# Autodesk Inventor assembly: Zusammenbau_Gruppe7
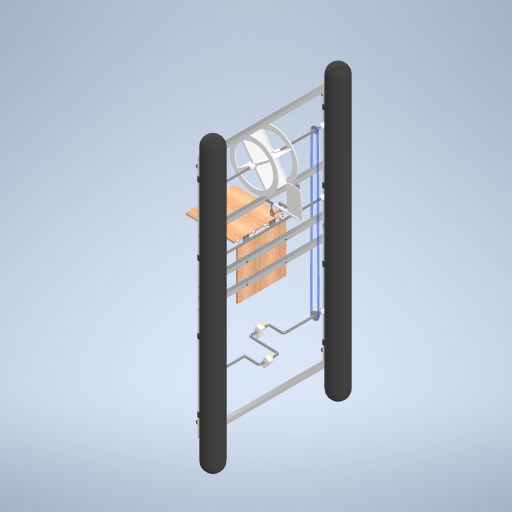
[picture p0: Inventor's stored thumbnail of the model, 512x512]
Saved by Autodesk Inventor 2024.4 (Build 284460000, 460)
## iProperties
Created: 2026-01-14
Part Number: Zusammenbau_Gruppe7
Description: Zusammenbau
Document SubType Name: Assembly
Designer: Philf
Mass: 49081.2 g
Surface Area: 141619 cm^2
Volume: 28441.6 cm^3
Density: 1.72568 g/cm^3
Masse[kg]: 49,1 kg
## Documents named in this file (35)
- C:\Users\Philf\Documents\Vault\Daten\I60-Konstruktion\I60-Gruppe-7\Konzept\Teil2\Zusammenbau_Gruppe7.iam
- C:\Users\Philf\Documents\Vault\Daten\I60-Konstruktion\I60-Gruppe-7\Gestell\Gestell_zsm.iam
- C:\Users\Philf\Documents\Vault\Daten\I60-Konstruktion\I60-Gruppe-7\Schwimmkoerper\Schwimmkoerper.iam
- C:\Users\Philf\Documents\Vault\Daten\I60-Konstruktion\I60-Gruppe-7\schaufelrad\Schaufelrad.iam
- C:\Users\Philf\Documents\Vault\Daten\I60-Konstruktion\I60-Gruppe-7\Tritt\Stange.iam
- C:\Users\Philf\Documents\Vault\Daten\I60-Konstruktion\I60-Gruppe-7\Tritt\Pedale.iam
- C:\Users\Philf\Documents\Vault\Daten\I60-Konstruktion\I60-Gruppe-7\Sitz\sitz_zusammenbau.iam
- C:\Users\Philf\Documents\Vault\Normteile\de-DE\DIN EN ISO 4032\DIN EN ISO 4032 - M10.ipt
- C:\Users\Philf\Documents\Vault\Normteile\de-DE\ISO 10642(2)\ISO 10642  - M10  x  70.ipt
- C:\Users\Philf\Documents\Vault\Daten\I60-Konstruktion\I60-Gruppe-7\Tritt\stopper2.ipt
- C:\Users\Philf\Documents\Vault\Normteile\de-DE\ISO 4762(1)\DIN EN ISO 4762 - M5 x 20.ipt
- C:\Users\Philf\Documents\Vault\Daten\I60-Konstruktion\I60-Gruppe-7\Tritt\6799K141_Machinable-Bore Corrosion-Resistant Sprocket.ipt
- C:\Users\Philf\Documents\Vault\Normteile\de-DE\ISO 4762(1)\DIN EN ISO 4762 - M10 x 60.ipt
- C:\Users\Philf\Documents\Vault\Normteile\de-DE\ISO 4762(1)\DIN EN ISO 4762 - M5 x 16.ipt
- C:\Users\Philf\Documents\Vault\Daten\I60-Konstruktion\I60-Gruppe-7\Tritt\6799K144_Machinable-Bore Corrosion-Resistant Sprocket\6799K144_Machinable-Bore Corrosion-Resistant Sprocket\6799K144_Machinable-Bore Corr.ipt
- C:\Users\Philf\Documents\Vault\Daten\I60-Konstruktion\I60-Gruppe-7\Zusammenbau\Konstruktions-Assistent\HTW-000642.iam
- C:\Users\Philf\Documents\Vault\Daten\I60-Konstruktion\I60-Gruppe-7\schaufelrad\Stangeschaufelrad.ipt
- C:\Users\Philf\Documents\Vault\Daten\I60-Konstruktion\I60-Gruppe-7\Steuern\HTW-000654.ipt
- C:\Users\Philf\Documents\Vault\Daten\I60-Konstruktion\I60-Gruppe-7\Steuern\Verbindung.ipt
- C:\Users\Philf\Documents\Vault\Daten\I60-Konstruktion\I60-Gruppe-7\Steuern\ustück.ipt
- C:\Users\Philf\Documents\Vault\Daten\I60-Konstruktion\I60-Gruppe-7\Steuern\clevisPin30.ipt
- C:\Users\Philf\Documents\Vault\Daten\I60-Konstruktion\I60-Gruppe-7\Steuern\cotterpin.ipt
- C:\Users\Philf\Documents\Vault\Daten\I60-Konstruktion\I60-Gruppe-7\Steuern\HTW-000679.ipt
- C:\Users\Philf\Documents\Vault\Daten\I60-Konstruktion\I60-Gruppe-7\Steuern\HTW-000681.ipt
- C:\Users\Philf\Documents\Vault\Daten\I60-Konstruktion\I60-Gruppe-7\Steuern\Rod End Nuts.ipt
- C:\Users\Philf\Documents\Vault\Daten\I60-Konstruktion\I60-Gruppe-7\Steuern\steuerstange.ipt
- C:\Users\Philf\Documents\Vault\Daten\I60-Konstruktion\I60-Gruppe-7\Steuern\HTW-000692.ipt
- C:\Users\Philf\Documents\Vault\Daten\I60-Konstruktion\I60-Gruppe-7\Gestell\richtungstange.ipt
- C:\Users\Philf\Documents\Vault\Daten\I60-Konstruktion\I60-Gruppe-7\Steuern\HTW-000702.ipt
- C:\Users\Philf\Documents\Vault\Normteile\de-DE\DIN EN ISO 7093-1\DIN EN ISO 7093-1 - 8.ipt
- C:\Users\Philf\Documents\Vault\Daten\I60-Konstruktion\I60-Gruppe-7\Gestell\LagerBund.ipt
- C:\Users\Philf\Documents\Vault\Normteile\de-DE\ISO 4762(1)\DIN EN ISO 4762 - M8 x 16.ipt
- C:\Users\Philf\Documents\Vault\Normteile\de-DE\ISO 4762(1)\DIN EN ISO 4762 - M8 x 25.ipt
- C:\Users\Philf\Documents\Vault\Normteile\de-DE\ISO 4762(1)\DIN EN ISO 4762 - M5 x 25.ipt
- C:\Users\Philf\Documents\Vault\Normteile\de-DE\ISO 4762(1)\DIN EN ISO 4762 - M5 x 8.ipt
## Components (98 placed, 34 different names)
1. Gestell_zsm:1 [sub-assembly] — Passend:1, Passend:2, Passend:3, Passend:4, Passend:5, Passend:6, Passend:7, Passend:8, Passend:9, Drehbar:1, Drehbar:4, Passend:12, Passend:13, Passend:14, Einfügen:1, Einfügen:2, Einfügen:3, Einfügen:4, Passend:24, Passend:26, Einfügen:9, Einfügen:10, Einfügen:11, Einfügen:12, Einfügen:13, Einfügen:14, Einfügen:15, Einfügen:16, Einfügen:17, Einfügen:18, Einfügen:19, Einfügen:20, Einfügen:29, Einfügen:30, Einfügen:31, Einfügen:32, Einfügen:33, Einfügen:34, Einfügen:35, Einfügen:36, Einfügen:37, Einfügen:38, Einfügen:39, Einfügen:40, Fluchtend:2, Passend:32, Fluchtend:3, Passend:70, Passend:74, Fluchtend:5, Passend:75, Passend:102, Passend:104, Einfügen:55, Einfügen:56
2. Schwimmkoerper:1 [sub-assembly] — Passend:5, Passend:7, Passend:8, Winkel:1
3. Schwimmkoerper:2 [sub-assembly] — Passend:4, Passend:6, Passend:9, Winkel:2, Fluchtend:2
4. Schaufelrad:1 [sub-assembly] — Drehbar:4, Passend:23, Passend:25, Winkel:3, Winkel:4, Passend:27, Passend:29
5. Stange:1 [sub-assembly] — Drehbar:1, Drehbar:2, Drehbar:3, Passend:10, Passend:11, Einfügen:21, Einfügen:22, Einfügen:23, Einfügen:24, Passend:30, Passend:31, Winkel:5
6. Pedale:1 [sub-assembly] — Drehbar:2, Passend:10
7. Pedale:2 [sub-assembly] — Drehbar:3, Passend:11
8. sitz_zusammenbau:1 [sub-assembly] — Passend:12, Passend:13, Passend:14, Passend:15, Passend:16, Passend:17, Passend:18
9. DIN EN ISO 4032 M10:1 — Einfügen:1
10. DIN EN ISO 4032 M10:2 — Einfügen:2
11. DIN EN ISO 4032 M10:3 — Einfügen:3
12. DIN EN ISO 4032 M10:4 — Einfügen:4
13. DIN EN ISO 10642 M10  x  70:1 — Passend:15
14. DIN EN ISO 10642 M10  x  70:2 — Passend:16
15. DIN EN ISO 10642 M10  x  70:3 — Passend:17
16. DIN EN ISO 10642 M10  x  70:4 — Passend:18
17. stopper2:1 — Passend:23, Passend:24, Winkel:4, Einfügen:5, Einfügen:6
18. stopper2:2 — Passend:25, Passend:26, Winkel:3, Einfügen:7, Einfügen:8
19. DIN EN ISO 4762 M5 x 20:1 — Einfügen:5
20. DIN EN ISO 4762 M5 x 20:2 — Einfügen:6
21. DIN EN ISO 4762 M5 x 20:3 — Einfügen:7
22. DIN EN ISO 4762 M5 x 20:4 — Einfügen:8
23. 6799K141_Machinable-Bore Corrosion-Resistant Sprocket:1 — Passend:27, Passend:29, Einfügen:28, Fluchtend:1, Drehung:1
24. DIN EN ISO 4762 M10 x 60:1 — Einfügen:9
25. DIN EN ISO 4762 M10 x 60:2 — Einfügen:10
26. DIN EN ISO 4762 M10 x 60:3 — Einfügen:11
27. DIN EN ISO 4762 M10 x 60:4 — Einfügen:12
28. DIN EN ISO 4762 M10 x 60:5 — Einfügen:13
29. DIN EN ISO 4762 M10 x 60:6 — Einfügen:14
30. DIN EN ISO 4762 M10 x 60:7 — Einfügen:15
31. DIN EN ISO 4762 M10 x 60:8 — Einfügen:16
32. DIN EN ISO 4762 M10 x 60:9 — Einfügen:17
33. DIN EN ISO 4762 M10 x 60:10 — Einfügen:18
34. DIN EN ISO 4762 M10 x 60:11 — Einfügen:19
35. DIN EN ISO 4762 M10 x 60:12 — Einfügen:20
36. DIN EN ISO 4762 M5 x 20:5 — Einfügen:21
37. DIN EN ISO 4762 M5 x 20:6 — Einfügen:22
38. DIN EN ISO 4762 M5 x 20:7 — Einfügen:23
39. DIN EN ISO 4762 M5 x 20:8 — Einfügen:24
40. DIN EN ISO 4762 M5 x 16:4 — Einfügen:28
41. DIN EN ISO 4032 M10:5 — Einfügen:29
42. DIN EN ISO 4032 M10:6 — Einfügen:30
43. DIN EN ISO 4032 M10:7 — Einfügen:31
44. DIN EN ISO 4032 M10:8 — Einfügen:32
45. DIN EN ISO 4032 M10:9 — Einfügen:33
46. DIN EN ISO 4032 M10:10 — Einfügen:34
47. DIN EN ISO 4032 M10:11 — Einfügen:35
48. DIN EN ISO 4032 M10:12 — Einfügen:36
49. DIN EN ISO 4032 M10:13 — Einfügen:37
50. DIN EN ISO 4032 M10:14 — Einfügen:38
51. DIN EN ISO 4032 M10:15 — Einfügen:39
52. DIN EN ISO 4032 M10:16 — Einfügen:40
53. 6799K144_Machinable-Bore Corr:1 — Passend:30, Passend:31, Fluchtend:1, Winkel:5, Drehung:1, Einfügen:41
54. Kettenantrieb:1 [sub-assembly]
55. DIN EN ISO 4762 M5 x 16:5 — Einfügen:41
56. Stangeschaufelrad:1 — Passend:32, Fluchtend:3, Passend:33, Passend:101, Passend:103
57. HTW-000654:1 — Passend:90, Passend:91, Fluchtend:11, Passend:105, Passend:106
58. Verbindung:1 — Passend:33, Passend:70, Einfügen:48, Einfügen:49, Einfügen:50, Fluchtend:11, Passend:105, Passend:106
59. ustück:1 — Passend:37, Passend:38, Passend:87, Passend:88, Passend:91
60. clevisPin30:1 — Passend:37, Passend:38, Passend:39, Passend:41, Passend:90
61. cotterpin:1 — Passend:39, Passend:41
62. ustück:2 — Passend:48, Passend:49, Passend:82, Passend:85, Passend:86
63. clevisPin30:2 — Passend:48, Passend:49, Passend:81
64. cotterpin:2
65. HTW-000681:1 — Passend:50, Passend:51, Passend:56, Passend:57, Passend:76, Passend:77, Passend:97, Fluchtend:9, Einfügen:43
66. Rod End Nuts:1 — Passend:50, Passend:51, Passend:81, Passend:82
67. ustück:3 — Passend:56, Passend:57, Passend:95
68. clevisPin30:3 — Passend:94
69. cotterpin:3
70. Rod End Nuts:2 — Passend:58, Passend:59, Passend:94, Passend:95
71. HTW-000679:2 — Passend:58, Passend:59, Passend:66, Passend:67
72. ustück:4 — Passend:68, Passend:69, Passend:93
73. clevisPin30:4 — Passend:92
74. cotterpin:4
75. Rod End Nuts:4 — Passend:66, Passend:67, Passend:92, Passend:93
76. steuerstange:1 — Passend:68, Passend:69, Passend:71, Passend:72, Passend:73, Passend:83, Passend:84, Passend:96, Fluchtend:10, Einfügen:42
77. HTW-000692:1 — Passend:71, Passend:72, Passend:73, Winkel:6, Einfügen:46, Einfügen:47
78. richtungstange:1 — Passend:74, Fluchtend:5, Passend:75, Passend:76, Passend:77, Passend:83, Passend:84, Passend:98, Passend:99
79. HTW-000702:1 — Passend:85, Passend:86, Passend:87, Passend:88
80. LagerBund:1 — Passend:97, Passend:98, Fluchtend:9
81. LagerBund:2 — Passend:96, Passend:99, Fluchtend:10
82. DIN EN ISO 7093-1 8:1 — Einfügen:42, Einfügen:45
83. DIN EN ISO 7093-1 8:2 — Einfügen:43, Einfügen:44
84. DIN EN ISO 4762 M8 x 16:1 — Einfügen:44
85. DIN EN ISO 4762 M8 x 16:2 — Einfügen:45
86. DIN EN ISO 4762 M8 x 25:1 — Einfügen:46
87. DIN EN ISO 4762 M8 x 25:2 — Einfügen:47
88. DIN EN ISO 4762 M5 x 25:1 — Einfügen:48
89. DIN EN ISO 4762 M5 x 8:1 — Einfügen:49
90. DIN EN ISO 4762 M5 x 8:2 — Einfügen:50
91. stopper2:3 — Passend:103, Passend:104, Einfügen:51, Einfügen:52
92. stopper2:4 — Passend:101, Passend:102, Einfügen:53, Einfügen:54
93. DIN EN ISO 4762 M5 x 20:9 — Einfügen:51
94. DIN EN ISO 4762 M5 x 20:10 — Einfügen:52
95. DIN EN ISO 4762 M5 x 20:11 — Einfügen:53
96. DIN EN ISO 4762 M5 x 20:12 — Einfügen:54
97. DIN EN ISO 4762 M10 x 60:13 — Einfügen:55
98. DIN EN ISO 4762 M10 x 60:14 — Einfügen:56
## Relationships (157: Mate 86, Insert 53, Flush 7, Angle 6, RevoluteJoint 4, RelateRotation 1)
- Passend:1 [Mate]: Gestell_zsm:1
- Passend:2 [Mate]: Gestell_zsm:1
- Passend:3 [Mate]: Gestell_zsm:1
- Passend:4 [Mate] (100 mm): Gestell_zsm:1 ↔ Schwimmkoerper:2
- Passend:5 [Mate] (100 mm): Gestell_zsm:1 ↔ Schwimmkoerper:1
- Passend:6 [Mate] (150 mm): Gestell_zsm:1 ↔ Schwimmkoerper:2
- Passend:7 [Mate] (150 mm): Gestell_zsm:1 ↔ Schwimmkoerper:1
- Passend:8 [Mate] (-18 mm): Gestell_zsm:1 ↔ Schwimmkoerper:1
- Passend:9 [Mate] (-22 mm): Gestell_zsm:1 ↔ Schwimmkoerper:2
- Winkel:1 [Angle] (90 deg): Schwimmkoerper:1
- Winkel:2 [Angle] (90 deg): Schwimmkoerper:2
- Drehbar:1 [RevoluteJoint] (-40 mm): Gestell_zsm:1 ↔ Stange:1
- Drehbar:2 [RevoluteJoint]: Stange:1 ↔ Pedale:1
- Drehbar:3 [RevoluteJoint] (-20 mm): Stange:1 ↔ Pedale:2
- Passend:10 [Mate]: Stange:1 ↔ Pedale:1
- Passend:11 [Mate]: Stange:1 ↔ Pedale:2
- Drehbar:4 [RevoluteJoint] (-40 mm): Gestell_zsm:1 ↔ Schaufelrad:1
- Passend:12 [Mate]: Gestell_zsm:1 ↔ sitz_zusammenbau:1
- Passend:13 [Mate]: Gestell_zsm:1 ↔ sitz_zusammenbau:1
- Passend:14 [Mate]: Gestell_zsm:1 ↔ sitz_zusammenbau:1
- Einfügen:1 [Insert]: Gestell_zsm:1 ↔ DIN EN ISO 4032 M10:1
- Einfügen:2 [Insert]: Gestell_zsm:1 ↔ DIN EN ISO 4032 M10:2
- Einfügen:3 [Insert]: Gestell_zsm:1 ↔ DIN EN ISO 4032 M10:3
- Einfügen:4 [Insert]: Gestell_zsm:1 ↔ DIN EN ISO 4032 M10:4
- Passend:15 [Mate]: sitz_zusammenbau:1 ↔ DIN EN ISO 10642 M10  x  70:1
- Passend:16 [Mate]: sitz_zusammenbau:1 ↔ DIN EN ISO 10642 M10  x  70:2
- Passend:17 [Mate]: sitz_zusammenbau:1 ↔ DIN EN ISO 10642 M10  x  70:3
- Passend:18 [Mate]: sitz_zusammenbau:1 ↔ DIN EN ISO 10642 M10  x  70:4
- Passend:23 [Mate]: Schaufelrad:1 ↔ stopper2:1
- Passend:24 [Mate]: Gestell_zsm:1 ↔ stopper2:1
- Passend:25 [Mate]: Schaufelrad:1 ↔ stopper2:2
- Passend:26 [Mate]: Gestell_zsm:1 ↔ stopper2:2
- Winkel:3 [Angle] (0 deg): Schaufelrad:1 ↔ stopper2:2
- Winkel:4 [Angle] (0 deg): Schaufelrad:1 ↔ stopper2:1
- Einfügen:5 [Insert]: stopper2:1 ↔ DIN EN ISO 4762 M5 x 20:1
- Einfügen:6 [Insert]: stopper2:1 ↔ DIN EN ISO 4762 M5 x 20:2
- Einfügen:7 [Insert]: stopper2:2 ↔ DIN EN ISO 4762 M5 x 20:3
- Einfügen:8 [Insert]: stopper2:2 ↔ DIN EN ISO 4762 M5 x 20:4
- Passend:27 [Mate]: Schaufelrad:1 ↔ 6799K141_Machinable-Bore Corrosion-Resistant Sprocket:1
- Passend:29 [Mate]: Schaufelrad:1 ↔ 6799K141_Machinable-Bore Corrosion-Resistant Sprocket:1
- Einfügen:9 [Insert]: Gestell_zsm:1 ↔ DIN EN ISO 4762 M10 x 60:1
- Einfügen:10 [Insert]: Gestell_zsm:1 ↔ DIN EN ISO 4762 M10 x 60:2
- Einfügen:11 [Insert]: Gestell_zsm:1 ↔ DIN EN ISO 4762 M10 x 60:3
- Einfügen:12 [Insert]: Gestell_zsm:1 ↔ DIN EN ISO 4762 M10 x 60:4
- Einfügen:13 [Insert]: Gestell_zsm:1 ↔ DIN EN ISO 4762 M10 x 60:5
- Einfügen:14 [Insert]: Gestell_zsm:1 ↔ DIN EN ISO 4762 M10 x 60:6
- Einfügen:15 [Insert]: Gestell_zsm:1 ↔ DIN EN ISO 4762 M10 x 60:7
- Einfügen:16 [Insert]: Gestell_zsm:1 ↔ DIN EN ISO 4762 M10 x 60:8
- Einfügen:17 [Insert]: Gestell_zsm:1 ↔ DIN EN ISO 4762 M10 x 60:9
- Einfügen:18 [Insert]: Gestell_zsm:1 ↔ DIN EN ISO 4762 M10 x 60:10
- Einfügen:19 [Insert]: Gestell_zsm:1 ↔ DIN EN ISO 4762 M10 x 60:11
- Einfügen:20 [Insert]: Gestell_zsm:1 ↔ DIN EN ISO 4762 M10 x 60:12
- Einfügen:21 [Insert]: Stange:1 ↔ DIN EN ISO 4762 M5 x 20:5
- Einfügen:22 [Insert]: Stange:1 ↔ DIN EN ISO 4762 M5 x 20:6
- Einfügen:23 [Insert]: Stange:1 ↔ DIN EN ISO 4762 M5 x 20:7
- Einfügen:24 [Insert]: Stange:1 ↔ DIN EN ISO 4762 M5 x 20:8
- Einfügen:28 [Insert]: 6799K141_Machinable-Bore Corrosion-Resistant Sprocket:1 ↔ DIN EN ISO 4762 M5 x 16:4
- Einfügen:29 [Insert]: Gestell_zsm:1 ↔ DIN EN ISO 4032 M10:5
- Einfügen:30 [Insert]: Gestell_zsm:1 ↔ DIN EN ISO 4032 M10:6
- Einfügen:31 [Insert]: Gestell_zsm:1 ↔ DIN EN ISO 4032 M10:7
- Einfügen:32 [Insert]: Gestell_zsm:1 ↔ DIN EN ISO 4032 M10:8
- Einfügen:33 [Insert]: Gestell_zsm:1 ↔ DIN EN ISO 4032 M10:9
- Einfügen:34 [Insert]: Gestell_zsm:1 ↔ DIN EN ISO 4032 M10:10
- Einfügen:35 [Insert]: Gestell_zsm:1 ↔ DIN EN ISO 4032 M10:11
- Einfügen:36 [Insert]: Gestell_zsm:1 ↔ DIN EN ISO 4032 M10:12
- Einfügen:37 [Insert]: Gestell_zsm:1 ↔ DIN EN ISO 4032 M10:13
- Einfügen:38 [Insert]: Gestell_zsm:1 ↔ DIN EN ISO 4032 M10:14
- Einfügen:39 [Insert]: Gestell_zsm:1 ↔ DIN EN ISO 4032 M10:15
- Einfügen:40 [Insert]: Gestell_zsm:1 ↔ DIN EN ISO 4032 M10:16
- Passend:30 [Mate]: Stange:1 ↔ 6799K144_Machinable-Bore Corr:1
- Passend:31 [Mate] (30 mm): Stange:1 ↔ 6799K144_Machinable-Bore Corr:1
- Fluchtend:1 [Flush]: 6799K141_Machinable-Bore Corrosion-Resistant Sprocket:1 ↔ 6799K144_Machinable-Bore Corr:1
- Winkel:5 [Angle] (0 deg): Stange:1 ↔ 6799K144_Machinable-Bore Corr:1
- Drehung:1 [RelateRotation] (1.2 ul): 6799K141_Machinable-Bore Corrosion-Resistant Sprocket:1 ↔ 6799K144_Machinable-Bore Corr:1
- Einfügen:41 [Insert]: 6799K144_Machinable-Bore Corr:1 ↔ DIN EN ISO 4762 M5 x 16:5
- Fluchtend:2 [Flush]: Gestell_zsm:1 ↔ Schwimmkoerper:2
- Passend:32 [Mate]: Gestell_zsm:1 ↔ Stangeschaufelrad:1
- Fluchtend:3 [Flush]: Gestell_zsm:1 ↔ Stangeschaufelrad:1
- Passend:33 [Mate]: Stangeschaufelrad:1 ↔ Verbindung:1
- Passend:37 [Mate]: ustück:1 ↔ clevisPin30:1
- Passend:38 [Mate]: ustück:1 ↔ clevisPin30:1
- Passend:39 [Mate]: clevisPin30:1 ↔ cotterpin:1
- Passend:41 [Mate] (-24 mm): clevisPin30:1 ↔ cotterpin:1
- [Mate]: clevisPin30:2 ↔ cotterpin:2
- [Mate] (-24 mm): clevisPin30:2 ↔ cotterpin:2
- Passend:48 [Mate]: ustück:2 ↔ clevisPin30:2
- Passend:49 [Mate]: ustück:2 ↔ clevisPin30:2
- Passend:50 [Mate]: HTW-000681:1 ↔ Rod End Nuts:1
- Passend:51 [Mate] (-10 mm): HTW-000681:1 ↔ Rod End Nuts:1
- [Mate]: clevisPin30:3 ↔ cotterpin:3
- [Mate] (-24 mm): clevisPin30:3 ↔ cotterpin:3
- [Mate]: ustück:3 ↔ clevisPin30:3
- [Mate]: ustück:3 ↔ clevisPin30:3
- Passend:56 [Mate]: HTW-000681:1 ↔ ustück:3
- Passend:57 [Mate] (-10 mm): HTW-000681:1 ↔ ustück:3
- Passend:58 [Mate]: Rod End Nuts:2 ↔ HTW-000679:2
- Passend:59 [Mate] (-8 mm): Rod End Nuts:2 ↔ HTW-000679:2
- [Mate]: clevisPin30:4 ↔ cotterpin:4
- [Mate] (-24 mm): clevisPin30:4 ↔ cotterpin:4
- [Mate]: ustück:4 ↔ clevisPin30:4
- [Mate]: ustück:4 ↔ clevisPin30:4
- Passend:66 [Mate]: HTW-000679:2 ↔ Rod End Nuts:4
- Passend:67 [Mate] (-8 mm): HTW-000679:2 ↔ Rod End Nuts:4
- Passend:68 [Mate]: ustück:4 ↔ steuerstange:1
- Passend:69 [Mate] (-10 mm): ustück:4 ↔ steuerstange:1
- Passend:70 [Mate] (300 mm): Gestell_zsm:1 ↔ Verbindung:1
- Passend:71 [Mate]: steuerstange:1 ↔ HTW-000692:1
- Passend:72 [Mate]: steuerstange:1 ↔ HTW-000692:1
- Passend:73 [Mate]: steuerstange:1 ↔ HTW-000692:1
- Passend:74 [Mate]: Gestell_zsm:1 ↔ richtungstange:1
- Fluchtend:5 [Flush]: Gestell_zsm:1 ↔ richtungstange:1
- Passend:75 [Mate] (410 mm): Gestell_zsm:1 ↔ richtungstange:1
- Passend:76 [Mate]: HTW-000681:1 ↔ richtungstange:1
- Passend:77 [Mate]: HTW-000681:1 ↔ richtungstange:1
- Passend:81 [Mate]: clevisPin30:2 ↔ Rod End Nuts:1
- Passend:82 [Mate]: ustück:2 ↔ Rod End Nuts:1
- Passend:83 [Mate]: steuerstange:1 ↔ richtungstange:1
- Passend:84 [Mate]: steuerstange:1 ↔ richtungstange:1
- Passend:85 [Mate]: ustück:2 ↔ HTW-000702:1
- Passend:86 [Mate] (-8 mm): ustück:2 ↔ HTW-000702:1
- Passend:87 [Mate]: ustück:1 ↔ HTW-000702:1
- Passend:88 [Mate] (-8 mm): ustück:1 ↔ HTW-000702:1
- Passend:90 [Mate]: HTW-000654:1 ↔ clevisPin30:1
- Passend:91 [Mate] (10 mm): HTW-000654:1 ↔ ustück:1
- Winkel:6 [Angle] (90 deg): HTW-000692:1
- Passend:92 [Mate]: clevisPin30:4 ↔ Rod End Nuts:4
- Passend:93 [Mate] (5 mm): ustück:4 ↔ Rod End Nuts:4
- Passend:94 [Mate]: clevisPin30:3 ↔ Rod End Nuts:2
- Passend:95 [Mate] (5 mm): ustück:3 ↔ Rod End Nuts:2
- Passend:96 [Mate]: steuerstange:1 ↔ LagerBund:2
- Passend:97 [Mate]: HTW-000681:1 ↔ LagerBund:1
- Passend:98 [Mate]: richtungstange:1 ↔ LagerBund:1
- Passend:99 [Mate]: richtungstange:1 ↔ LagerBund:2
- Fluchtend:9 [Flush]: HTW-000681:1 ↔ LagerBund:1
- Fluchtend:10 [Flush]: steuerstange:1 ↔ LagerBund:2
- Einfügen:42 [Insert]: steuerstange:1 ↔ DIN EN ISO 7093-1 8:1
- Einfügen:43 [Insert]: HTW-000681:1 ↔ DIN EN ISO 7093-1 8:2
- Einfügen:44 [Insert]: DIN EN ISO 7093-1 8:2 ↔ DIN EN ISO 4762 M8 x 16:1
- Einfügen:45 [Insert]: DIN EN ISO 7093-1 8:1 ↔ DIN EN ISO 4762 M8 x 16:2
- Einfügen:46 [Insert]: HTW-000692:1 ↔ DIN EN ISO 4762 M8 x 25:1
- Einfügen:47 [Insert]: HTW-000692:1 ↔ DIN EN ISO 4762 M8 x 25:2
- Einfügen:48 [Insert]: Verbindung:1 ↔ DIN EN ISO 4762 M5 x 25:1
- Einfügen:49 [Insert]: Verbindung:1 ↔ DIN EN ISO 4762 M5 x 8:1
- Einfügen:50 [Insert]: Verbindung:1 ↔ DIN EN ISO 4762 M5 x 8:2
- Fluchtend:11 [Flush] (-40 mm): HTW-000654:1 ↔ Verbindung:1
- Passend:101 [Mate]: Stangeschaufelrad:1 ↔ stopper2:4
- Passend:102 [Mate]: Gestell_zsm:1 ↔ stopper2:4
- Passend:103 [Mate]: Stangeschaufelrad:1 ↔ stopper2:3
- Passend:104 [Mate]: Gestell_zsm:1 ↔ stopper2:3
- Einfügen:51 [Insert]: stopper2:3 ↔ DIN EN ISO 4762 M5 x 20:9
- Einfügen:52 [Insert]: stopper2:3 ↔ DIN EN ISO 4762 M5 x 20:10
- Einfügen:53 [Insert]: stopper2:4 ↔ DIN EN ISO 4762 M5 x 20:11
- Einfügen:54 [Insert]: stopper2:4 ↔ DIN EN ISO 4762 M5 x 20:12
- Einfügen:55 [Insert]: Gestell_zsm:1 ↔ DIN EN ISO 4762 M10 x 60:13
- Einfügen:56 [Insert]: Gestell_zsm:1 ↔ DIN EN ISO 4762 M10 x 60:14
- Passend:105 [Mate]: HTW-000654:1 ↔ Verbindung:1
- Passend:106 [Mate]: HTW-000654:1 ↔ Verbindung:1
## Named parameters: d236_d229 = 0 mm, d237_d231 = -24 mm, d265_d236_d229 = 0 mm, d266_d237_d231 = -24 mm, d267_d238 = 0 mm, d268_d239 = 0 mm, d279_d265_d236_d229 = 0 mm, d280_d266_d237_d231 = -24 mm, d281_d267_d238 = 0 mm, d282_d268_d239 = 0 mm
